# Autodesk Inventor assembly: Sestava TF-Luna a držáku
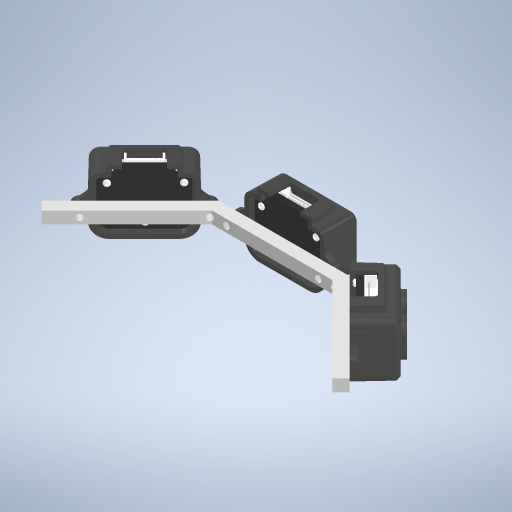
[picture p0: Inventor's stored thumbnail of the model, 512x512]
Saved by Autodesk Inventor 2024 (Build 280153000, 153)
## iProperties
Created: 2023-11-01
Part Number: Sestava TF-Luna a držáku
Document SubType Name: Assembly
Designer: 42060
Author: 42060
## Documents named in this file (3)
- C:\Users\42060\Desktop\ŠKOLA\Mini sumo\RoboCop\- 3D -\wip\Sestava TF-Luna a držáku.iam
- C:\Users\42060\Desktop\ŠKOLA\Mini sumo\RoboCop\- 3D -\el._parts\AssemBeneWake TF-LUNA.ipt
- C:\Users\42060\Desktop\ŠKOLA\Mini sumo\RoboCop\- 3D -\wip\Držák TF-Luna.ipt
## Components (4 placed, 2 different names)
1. AssemBeneWake TF-LUNA:1 — Vložit:1, Vložit:2
2. AssemBeneWake TF-LUNA:2 — Tuhé:1
3. AssemBeneWake TF-LUNA:3 — Tuhé:2
4. Držák TF-Luna:1 — Vložit:1, Vložit:2, Tuhé:1, Tuhé:2
## Relationships (4: Insert 2, WeldJoint 2)
- Vložit:1 [Insert]: AssemBeneWake TF-LUNA:1 ↔ Držák TF-Luna:1
- Vložit:2 [Insert]: AssemBeneWake TF-LUNA:1 ↔ Držák TF-Luna:1
- Tuhé:1 [WeldJoint]: AssemBeneWake TF-LUNA:2 ↔ Držák TF-Luna:1
- Tuhé:2 [WeldJoint]: AssemBeneWake TF-LUNA:3 ↔ Držák TF-Luna:1
